# Autodesk Inventor assembly: Obudowa
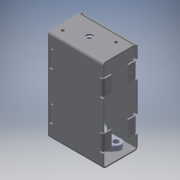
[picture p0: Inventor's stored thumbnail of the model, 180x180]
Saved by Autodesk Inventor 2019.4 (Build 234330000, 330)
## iProperties
Created: 2020-08-21
Part Number: Obudowa
Material: Ogólny
Document SubType Name: Assembly
Designer: barto
Author: barto
## Documents named in this file (4)
- F:\MUM\Obudowa.iam
- F:\MUM\GlownaObudowa.ipt
- C:\Users\barto\OneDrive\Pulpit\UCFL-201.ipt
- F:\MUM\ZaslepkaObudowa.ipt
## Components (4 placed, 3 different names)
1. GlownaObudowa:1 — Zestawiające:1, Zestawiające:2, Zestawiające:3, Zestawiające:4, Równoległe:1, Równoległe:2, Zestawiające:5, Zestawiające:6, Zestawiające:7
2. UCFL-201:1 — Zestawiające:1, Zestawiające:2, Zestawiające:3
3. ZaslepkaObudowa:1 — Zestawiające:4, Równoległe:1, Równoległe:2
4. UCFL-201:2 — Zestawiające:5, Zestawiające:6, Zestawiające:7
## Relationships (9: Mate 7, Flush 2)
- Zestawiające:1 [Mate]: GlownaObudowa:1 ↔ UCFL-201:1
- Zestawiające:2 [Mate]: GlownaObudowa:1 ↔ UCFL-201:1
- Zestawiające:3 [Mate]: GlownaObudowa:1 ↔ UCFL-201:1
- Zestawiające:4 [Mate]: GlownaObudowa:1 ↔ ZaslepkaObudowa:1
- Równoległe:1 [Flush]: GlownaObudowa:1 ↔ ZaslepkaObudowa:1
- Równoległe:2 [Flush]: GlownaObudowa:1 ↔ ZaslepkaObudowa:1
- Zestawiające:5 [Mate]: GlownaObudowa:1 ↔ UCFL-201:2
- Zestawiające:6 [Mate]: GlownaObudowa:1 ↔ UCFL-201:2
- Zestawiające:7 [Mate]: GlownaObudowa:1 ↔ UCFL-201:2
